# Autodesk Inventor assembly: Than+CB
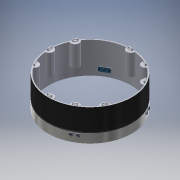
[picture p0: Inventor's stored thumbnail of the model, 180x180]
Saved by Autodesk Inventor 2019 (Build 230136000, 136)
## iProperties
Created: 2021-01-14
Part Number: Than+CB
Document SubType Name: Assembly
Designer: Admin
Author: Admin
## Documents named in this file (3)
- C:\Users\Admin\Documents\Inventor\Doan\Than+CB.iam
- C:\Users\Admin\Documents\Inventor\Doan\Than_new.ipt
- C:\Users\Admin\Documents\Inventor\Doan\HC-SR04.iam
## Components (5 placed, 2 different names)
1. Than_new:1 — Mate:1, Mate:2, Mate:3
2. HC-SR04:1 [sub-assembly] — Mate:1, Mate:2
3. HC-SR04:2 [sub-assembly]
4. HC-SR04:3 [sub-assembly]
5. HC-SR04:4 [sub-assembly] — Mate:3
## Component patterns: (4 elements, first: HC-SR04:1)
## Relationships (3: Mate 3)
- Mate:1: Than_new:1 ↔ HC-SR04:1
- Mate:2: Than_new:1 ↔ HC-SR04:1
- Mate:3: Than_new:1 ↔ HC-SR04:4
